# Autodesk Inventor assembly: ImmersionCuvetteAssembly
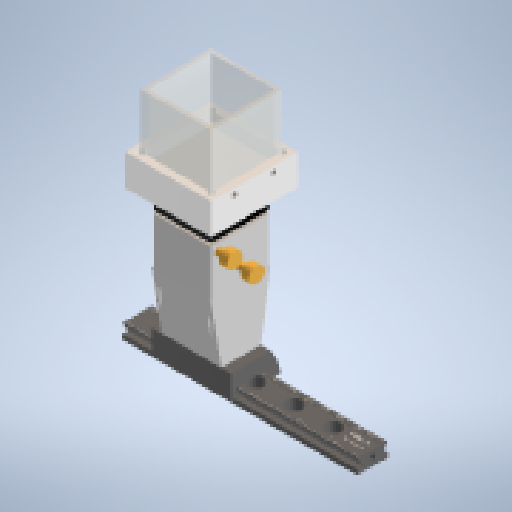
[picture p0: Inventor's stored thumbnail of the model, 512x512]
Saved by Autodesk Inventor 2023 (Build 270158000, 158)
## iProperties
Created: 2022-02-28
Part Number: ImmersionCuvetteAssembly
Document SubType Name: Assembly
Designer: nvladi
Author: nvladi
## Documents named in this file (8)
- C:\Users\Public\github\benchtop-hardware\Benchtop\custom-parts\sample_handling\immersion-chamber-mounting\ImmersionCuvetteAssembly.iam
- C:\Users\Public\github\benchtop-hardware\Benchtop\custom-parts\sample_handling\immersion-chamber-mounting\Large-cuvette-mount-40mm-V3.ipt
- C:\Users\Public\github\benchtop-hardware\Benchtop\CAD-model-Inventor\library\Portmann Instruments\UQ-753-40x40x45mm.ipt
- C:\Users\Public\github\benchtop-hardware\Benchtop\CAD-model-Inventor\library\Thorlabs\rails\RLA150_M.ipt
- C:\Users\Public\github\benchtop-hardware\Benchtop\CAD-model-Inventor\library\Thorlabs\rails\RC2_M.ipt
- C:\Users\Public\github\benchtop-hardware\Benchtop\custom-parts\sample_handling\immersion-chamber-mounting\RadianDyes-PDT(small)\RD-PDT-S-to-RC2-height40mm.ipt
- C:\Users\Public\github\benchtop-hardware\Benchtop\CAD-model-Inventor\library\Thorlabs\kinematic_bases\KB25_M-Step.ipt
- C:\Users\Public\github\benchtop-hardware\Benchtop\CAD-model-Inventor\library\RadiantDyes\RadiantDyes-RD-PDT-S(approx).ipt
## Components (7 placed, 7 different names)
1. Large-cuvette-mount-40mm-V3:1 — Mate:7, Mate:8, Mate:11, Mate:12, Mate:13
2. UQ-753-40x40x45mm:1 — Mate:11, Mate:12, Mate:13
3. RLA150_M:1 — Mate:4, Flush:1
4. RC2_M:1 — Mate:4, Flush:1, Mate:5, Mate:6, Flush:3
5. RD-PDT-S-to-RC2-height40mm:2 — Mate:5, Mate:6, Mate:9, Flush:2
6. KB25_M-Step:1 — Mate:7, Mate:8, Mate:10, Insert:1
7. RadiantDyes-RD-PDT-S(approx):1 — Mate:9, Flush:2, Flush:3, Mate:10, Insert:1
## Relationships (14: Mate 10, Flush 3, Insert 1)
- Mate:4: RLA150_M:1 ↔ RC2_M:1
- Flush:1 (-3.2 mm): RLA150_M:1 ↔ RC2_M:1
- Mate:5: RC2_M:1 ↔ RD-PDT-S-to-RC2-height40mm:2
- Mate:6: RC2_M:1 ↔ RD-PDT-S-to-RC2-height40mm:2
- Mate:7: Large-cuvette-mount-40mm-V3:1 ↔ KB25_M-Step:1
- Mate:8: Large-cuvette-mount-40mm-V3:1 ↔ KB25_M-Step:1
- Mate:9: RD-PDT-S-to-RC2-height40mm:2 ↔ RadiantDyes-RD-PDT-S(approx):1
- Flush:2: RD-PDT-S-to-RC2-height40mm:2 ↔ RadiantDyes-RD-PDT-S(approx):1
- Flush:3 (-6.3 mm): RC2_M:1 ↔ RadiantDyes-RD-PDT-S(approx):1
- Mate:10: KB25_M-Step:1 ↔ RadiantDyes-RD-PDT-S(approx):1
- Insert:1: KB25_M-Step:1 ↔ RadiantDyes-RD-PDT-S(approx):1
- Mate:11: Large-cuvette-mount-40mm-V3:1 ↔ UQ-753-40x40x45mm:1
- Mate:12: Large-cuvette-mount-40mm-V3:1 ↔ UQ-753-40x40x45mm:1
- Mate:13: Large-cuvette-mount-40mm-V3:1 ↔ UQ-753-40x40x45mm:1
